# Autodesk Inventor assembly: Full Robot
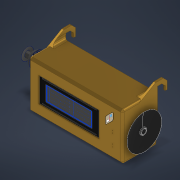
[picture p0: Inventor's stored thumbnail of the model, 180x180]
Saved by Autodesk Inventor 2022 (Build 260153000, 153)
## iProperties
Created: 2021-08-06
Part Number: Full Robot
Document SubType Name: Assembly
Designer: sidsa
Author: sidsa
## Documents named in this file (7)
- D:\My Documents\gitHUB Rocketry\mlh-robo-hacks\Inventor CAD\Full Robot.iam
- D:\My Documents\gitHUB Rocketry\mlh-robo-hacks\Inventor CAD\Electronics\20x4 LCD\ERM2004-2_3D.ipt
- D:\My Documents\gitHUB Rocketry\mlh-robo-hacks\Inventor CAD\Electronics\Joystick\Joystick HW504 Board.ipt
- D:\My Documents\gitHUB Rocketry\mlh-robo-hacks\Inventor CAD\Mount Case.ipt
- D:\My Documents\gitHUB Rocketry\mlh-robo-hacks\Inventor CAD\Electronics\Speaker\Speaker.ipt
- D:\My Documents\gitHUB Rocketry\mlh-robo-hacks\Inventor CAD\Electronics\Breadboard\MiniBreadboard.ipt
- D:\My Documents\gitHUB Rocketry\mlh-robo-hacks\Inventor CAD\Electronics\Arduino\Arduino_NANO_CH340.ipt
## Components (6 placed, 6 different names)
1. ERM2004-2_3D:1 — Mate:2
2. Joystick HW504 Board:1 — Mate:3
3. Mount Case:1 — Mate:2, Mate:3, Mate:7, Mate:8
4. Speaker:1 — Mate:7
5. MiniBreadboard:1 — Mate:8, Mate:9
6. Arduino_NANO_CH340:1 — Mate:9
## Relationships (5: Mate 5)
- Mate:2: ERM2004-2_3D:1 ↔ Mount Case:1
- Mate:3: Joystick HW504 Board:1 ↔ Mount Case:1
- Mate:7: Mount Case:1 ↔ Speaker:1
- Mate:8: Mount Case:1 ↔ MiniBreadboard:1
- Mate:9: MiniBreadboard:1 ↔ Arduino_NANO_CH340:1
